# Autodesk Inventor assembly: suspension_one_side
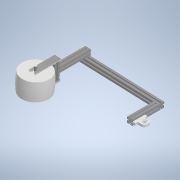
[picture p0: Inventor's stored thumbnail of the model, 180x180]
Saved by Autodesk Inventor 2021 (Build 250183000, 183)
## iProperties
Created: 2021-05-27
Part Number: suspension_one_side
Document SubType Name: Assembly
Designer: gisen
Author: gisen
## Documents named in this file (8)
- C:\Users\gisen\workspace\beetle_inventor_model\suspension\rocker_left.iam
- C:\Users\gisen\workspace\beetle_inventor_model\suspension\C-BGHKA6902ZZ-30\C-BGHKA6902ZZ-30.iam
- C:\Users\gisen\workspace\beetle_inventor_model\suspension\frame\AFS-3030-435.ipt
- C:\Users\gisen\workspace\beetle_inventor_model\suspension\frame\AFS-3030-200.ipt
- C:\Users\gisen\workspace\beetle_inventor_model\suspension\wheel_with_mounts.iam
- C:\Users\gisen\workspace\beetle_inventor_model\suspension\frame\AFS-3030-174.ipt
- C:\Users\gisen\workspace\beetle_inventor_model\suspension\CAM\rocker_frame_mount_00.ipt
- C:\Users\gisen\workspace\beetle_inventor_model\suspension\CAM\rocker_frame_mount_01.ipt
## Components (7 placed, 7 different names)
1. C-BGHKA6902ZZ-30:1 [sub-assembly] — メイト:5, メイト:18, フラッシュ:12
2. AFS-3030-435:1 — メイト:5, フラッシュ:6, フラッシュ:7, メイト:6, メイト:8, メイト:15, フラッシュ:9, フラッシュ:18, メイト:23, メイト:24
3. AFS-3030-174:1 — フラッシュ:6, フラッシュ:7, メイト:6, メイト:18, フラッシュ:12
4. rocker_frame_mount_00:1 — メイト:8, メイト:16, フラッシュ:18, フラッシュ:13, メイト:23
5. AFS-3030-200:1 — メイト:13, フラッシュ:8, メイト:14, メイト:15, フラッシュ:9, メイト:16, メイト:22
6. wheel_with_mounts:1 [sub-assembly] — メイト:13, フラッシュ:8, メイト:14, フラッシュ:10
7. rocker_frame_mount_01:1 — メイト:22, フラッシュ:13, メイト:24
## Relationships (19: Mate 11, Flush 8)
- メイト:5 [Mate] (-15 mm): C-BGHKA6902ZZ-30:1 ↔ AFS-3030-435:1
- フラッシュ:6 [Flush]: AFS-3030-435:1 ↔ AFS-3030-174:1
- フラッシュ:7 [Flush]: AFS-3030-435:1 ↔ AFS-3030-174:1
- メイト:6 [Mate]: AFS-3030-435:1 ↔ AFS-3030-174:1
- メイト:8 [Mate]: AFS-3030-435:1 ↔ rocker_frame_mount_00:1
- メイト:13 [Mate]: AFS-3030-200:1 ↔ wheel_with_mounts:1
- フラッシュ:8 [Flush]: AFS-3030-200:1 ↔ wheel_with_mounts:1
- メイト:14 [Mate]: AFS-3030-200:1 ↔ wheel_with_mounts:1
- メイト:15 [Mate] (3 mm): AFS-3030-435:1 ↔ AFS-3030-200:1
- フラッシュ:9 [Flush]: AFS-3030-435:1 ↔ AFS-3030-200:1
- メイト:16 [Mate]: rocker_frame_mount_00:1 ↔ AFS-3030-200:1
- フラッシュ:18 [Flush]: AFS-3030-435:1 ↔ rocker_frame_mount_00:1
- メイト:18 [Mate]: C-BGHKA6902ZZ-30:1 ↔ AFS-3030-174:1
- フラッシュ:10 [Flush]: wheel_with_mounts:1
- フラッシュ:12 [Flush]: C-BGHKA6902ZZ-30:1 ↔ AFS-3030-174:1
- メイト:22 [Mate]: AFS-3030-200:1 ↔ rocker_frame_mount_01:1
- フラッシュ:13 [Flush]: rocker_frame_mount_00:1 ↔ rocker_frame_mount_01:1
- メイト:23 [Mate]: AFS-3030-435:1 ↔ rocker_frame_mount_00:1
- メイト:24 [Mate]: AFS-3030-435:1 ↔ rocker_frame_mount_01:1
